# Autodesk Inventor assembly: cylinderAssemblyV4
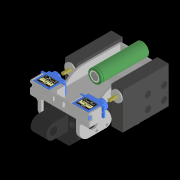
[picture p0: Inventor's stored thumbnail of the model, 180x180]
Saved by Autodesk Inventor 2021 (Build 250183000, 183)
## iProperties
Created: 2024-03-18
Part Number: cylinderAssemblyV4
Document SubType Name: Assembly
Designer: top10
Author: top10
## Documents named in this file (9)
- D:\Files\Graduation Project\V4_manfoulid\Workspaces\Workspace\cylinderAssemblyV4.iam
- D:\Files\Graduation Project\V4_manfoulid\Workspaces\Workspace\Hydr_CylinV4.ipt
- D:\Files\Graduation Project\V4_manfoulid\Workspaces\Workspace\BodyV4.iam
- D:\Files\Graduation Project\V4_manfoulid\Workspaces\Workspace\Val_BodV4_MLeft.ipt
- D:\Files\Graduation Project\V4_manfoulid\Workspaces\Workspace\SG90-servo-motor.ipt
- D:\Files\Graduation Project\V4_manfoulid\Workspaces\Workspace\MIR_Left\BodyV4_MIR_Left.iam
- D:\Files\Graduation Project\V4_manfoulid\Workspaces\Workspace\MIR_Left\SG90-servo-motor_MIR_Left.ipt
- D:\Files\Graduation Project\V4_manfoulid\Workspaces\Workspace\M_holder.ipt
- D:\Files\Graduation Project\V4_manfoulid\Workspaces\Workspace\18650 Li-Ion.ipt
## Components (8 placed, 8 different names)
1. Hydr_CylinV4:1 — Flush:1, Flush:2, Flush:3, Mate:1, Mate:2, Mate:3, Mate:4, Mate:5, Mate:6, Flush:4, Flush:5, Flush:6
2. BodyV4_Right:1 [sub-assembly] — Mate:1, Mate:2, Mate:3, Mate:7, Angle:1
3. Val_BodV4_MLeft:1 — Mate:4, Mate:5, Mate:6
4. SG90-servo-motor:1 — Mate:7, Angle:1, Flush:4
5. BodyV4_MIR_Left:1 [sub-assembly] — Angle:2, Mate:8
6. SG90-servo-motor_MIR_Left:1 — Angle:2, Mate:8
7. M_holder:1 — Flush:5, Flush:6
8. 18650 Li-Ion:1
## Relationships (16: Mate 8, Flush 6, Angle 2)
- Flush:1: Hydr_CylinV4:1
- Flush:2: Hydr_CylinV4:1
- Flush:3: Hydr_CylinV4:1
- Mate:1: Hydr_CylinV4:1 ↔ BodyV4_Right:1
- Mate:2: Hydr_CylinV4:1 ↔ BodyV4_Right:1
- Mate:3: Hydr_CylinV4:1 ↔ BodyV4_Right:1
- Mate:4: Hydr_CylinV4:1 ↔ Val_BodV4_MLeft:1
- Mate:5: Hydr_CylinV4:1 ↔ Val_BodV4_MLeft:1
- Mate:6: Hydr_CylinV4:1 ↔ Val_BodV4_MLeft:1
- Mate:7: BodyV4_Right:1 ↔ SG90-servo-motor:1
- Angle:1 (0 deg): BodyV4_Right:1 ↔ SG90-servo-motor:1
- Flush:4: Hydr_CylinV4:1 ↔ SG90-servo-motor:1
- Angle:2 (0 deg): BodyV4_MIR_Left:1 ↔ SG90-servo-motor_MIR_Left:1
- Mate:8: BodyV4_MIR_Left:1 ↔ SG90-servo-motor_MIR_Left:1
- Flush:5: Hydr_CylinV4:1 ↔ M_holder:1
- Flush:6: Hydr_CylinV4:1 ↔ M_holder:1
